# Autodesk Inventor assembly: Assembly1
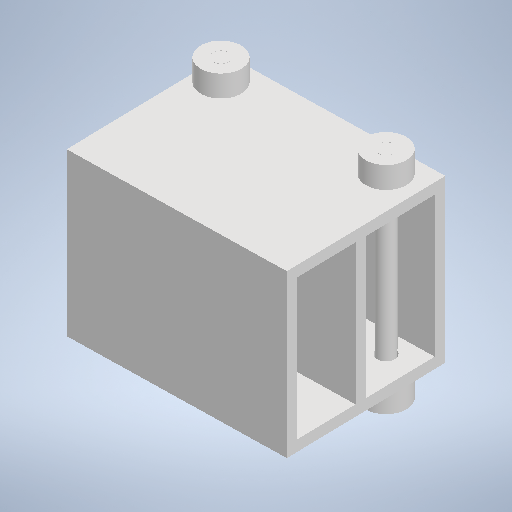
[picture p0: Inventor's stored thumbnail of the model, 512x512]
Saved by Autodesk Inventor 2025.3 (Build 293356030, 356C)
## iProperties
Created: 2026-06-23
Part Number: Assembly1
Document SubType Name: Assembly
Designer: user
Author: user
## Documents named in this file (4)
- C:\Docs\shcool\dojo\Boxed\Assembly1.iam
- C:\Docs\shcool\dojo\Boxed\body.ipt
- C:\Docs\shcool\dojo\Boxed\shaft.ipt
- C:\Docs\shcool\dojo\Boxed\wheel.ipt
## Components (7 placed, 3 different names)
1. body:1 — Insert:1, Insert:2
2. shaft:1 — Insert:1, Insert:4, Insert:6
3. wheel:1 — Insert:6
4. shaft:2 — Insert:2, Insert:3, Insert:5
5. wheel:2 — Insert:4
6. wheel:3 — Insert:5
7. wheel:4 — Insert:3
## Relationships (6: Insert 6)
- Insert:1 (50 mm): body:1 ↔ shaft:1
- Insert:2 (50 mm): body:1 ↔ shaft:2
- Insert:3: shaft:2 ↔ wheel:4
- Insert:4: shaft:1 ↔ wheel:2
- Insert:5: shaft:2 ↔ wheel:3
- Insert:6: shaft:1 ↔ wheel:1
